# Autodesk Inventor assembly: Assembly1
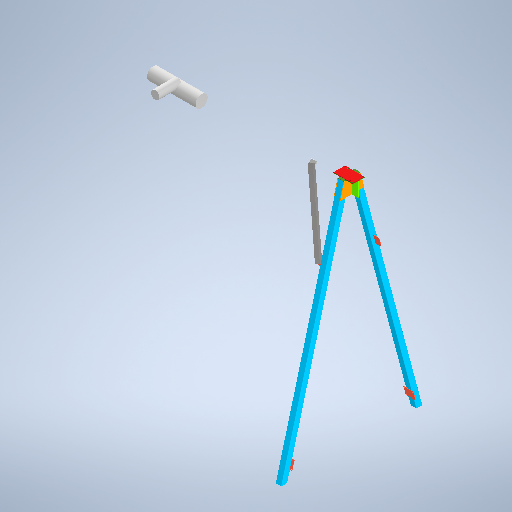
[picture p0: Inventor's stored thumbnail of the model, 512x512]
Saved by Autodesk Inventor 2025 (Build 290162010, 162A)
## iProperties
Created: 2024-06-11
Part Number: Assembly1
Document SubType Name: Assembly
Designer: admin
Author: admin
## Documents named in this file (8)
- C:\Users\pokla\Documents\Inventor\Goat\Goat-main\Assembly1.iam
- C:\Users\pokla\Documents\Inventor\Goat\Goat-main\WRS 000,000 кран козловой 6х4.ipt
- C:\Users\pokla\Documents\Inventor\Goat\Goat-main\Тельфер Таль электрическая.ipt
- C:\Users\pokla\Documents\Inventor\Goat\Goat-main\Сrane plate 1.ipt
- C:\Users\pokla\Documents\Inventor\Goat\Goat-main\Assembly2 стойка.iam
- C:\Users\pokla\Documents\Inventor\Goat\Goat-main\Сrane plate 5.1.ipt
- C:\Users\pokla\Documents\Inventor\Goat\Goat-main\JIS G 3192 - 100 x 50 x 5 - 1500 - 0,00936(4).ipt
- C:\Users\pokla\Documents\Inventor\Goat\Goat-main\Сrane plate 5.ipt
## Components (9 placed, 7 different names)
1. WRS 000,000 кран козловой 6х4.ipt:1 — Mate:2, Mate:3, Flush:3
2. Тельфер Таль электрическая.ipt:1 — Mate:4
3. Сrane plate 1.ipt:1 — Flush:18
4. Assembly2 стойка.iam:1 [sub-assembly] — Rotational:1, Mate:18, Rigid:3
5. Сrane plate 5.1.ipt:1 — Flush:24, Flush:25, Mate:16, Rotational:1, Mate:18
6. JIS G 3192 - 100 x 50 x 5 - 1500 - 0,00936(4).ipt:1 — Flush:24, Flush:25, Mate:16, Flush:26, Flush:27, Mate:17
7. Сrane plate 5.1.ipt:2 — Flush:26, Flush:27, Mate:17, Rotational:2, Mate:19
8. Сrane plate 5.ipt:1 — Rotational:2, Mate:19
9. Assembly2 стойка.iam:2 [sub-assembly] — Rigid:3
## Relationships (19: Flush 8, Mate 7, WeldJoint 2, RevoluteJoint 2)
- Mate:2: WRS 000,000 кран козловой 6х4.ipt:1
- Mate:3: WRS 000,000 кран козловой 6х4.ipt:1
- Flush:3: WRS 000,000 кран козловой 6х4.ipt:1
- Mate:4: Тельфер Таль электрическая.ipt:1
- [Flush]: Assembly2 стойка.iam:1
- Flush:18: Сrane plate 1.ipt:1
- [Flush]: Assembly2 стойка.iam:1
- [WeldJoint]: Сrane plate 1.ipt:1 ↔ Assembly2 стойка.iam:1
- Flush:24: Сrane plate 5.1.ipt:1 ↔ JIS G 3192 - 100 x 50 x 5 - 1500 - 0,00936(4).ipt:1
- Flush:25: Сrane plate 5.1.ipt:1 ↔ JIS G 3192 - 100 x 50 x 5 - 1500 - 0,00936(4).ipt:1
- Mate:16: Сrane plate 5.1.ipt:1 ↔ JIS G 3192 - 100 x 50 x 5 - 1500 - 0,00936(4).ipt:1
- Flush:26: JIS G 3192 - 100 x 50 x 5 - 1500 - 0,00936(4).ipt:1 ↔ Сrane plate 5.1.ipt:2
- Flush:27: JIS G 3192 - 100 x 50 x 5 - 1500 - 0,00936(4).ipt:1 ↔ Сrane plate 5.1.ipt:2
- Mate:17: JIS G 3192 - 100 x 50 x 5 - 1500 - 0,00936(4).ipt:1 ↔ Сrane plate 5.1.ipt:2
- Rotational:1 [RevoluteJoint]: Assembly2 стойка.iam:1 ↔ Сrane plate 5.1.ipt:1
- Mate:18: Assembly2 стойка.iam:1 ↔ Сrane plate 5.1.ipt:1
- Rotational:2 [RevoluteJoint]: Сrane plate 5.1.ipt:2 ↔ Сrane plate 5.ipt:1
- Mate:19: Сrane plate 5.1.ipt:2 ↔ Сrane plate 5.ipt:1
- Rigid:3 [WeldJoint]: Assembly2 стойка.iam:1 ↔ Assembly2 стойка.iam:2
